# Autodesk Inventor assembly: PitchAssembly
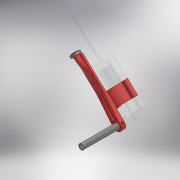
[picture p0: Inventor's stored thumbnail of the model, 180x180]
Saved by Autodesk Inventor 2018 (Build 220112000, 112)
## iProperties
Created: 2018-03-26
Part Number: PitchAssembly
Document SubType Name: Assembly
Designer: mansu
Author: mansu
## Documents named in this file (5)
- F:\OneDrive\Documents\2018 UBC\ELEC 391\Controller\cad\release\PitchAssemblyB.iam
- F:\OneDrive\Documents\2018 UBC\ELEC 391\Controller\cad\release\Rod3_8in.ipt
- F:\OneDrive\Documents\2018 UBC\ELEC 391\Controller\cad\release\PitchMotor\pitch_motor_flashlight_attached_model.iam
- F:\OneDrive\Documents\2018 UBC\ELEC 391\Controller\cad\release\R1038_ZZ_W Bearing.ipt
- F:\OneDrive\Documents\2018 UBC\ELEC 391\Controller\cad\release\ShaftArmB.ipt
## Components (4 placed, 4 different names)
1. Rod3_8in:1 — Mate:9, Mate:10, Flush:1
2. pitch_motor_flashlight_attached_model:1 [sub-assembly] — Mate:11
3. R1038_ZZ_W Bearing:1 — Mate:12, Flush:2
4. ShaftArmB:1 — Mate:10, Mate:11, Flush:1, Mate:12, Flush:2
## Relationships (6: Mate 4, Flush 2)
- Mate:9: Rod3_8in:1
- Mate:10: Rod3_8in:1 ↔ ShaftArmB:1
- Mate:11: pitch_motor_flashlight_attached_model:1 ↔ ShaftArmB:1
- Flush:1: Rod3_8in:1 ↔ ShaftArmB:1
- Mate:12: R1038_ZZ_W Bearing:1 ↔ ShaftArmB:1
- Flush:2 (1 mm): R1038_ZZ_W Bearing:1 ↔ ShaftArmB:1
